# Autodesk Inventor assembly: Estante
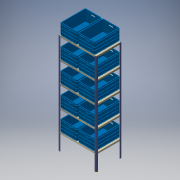
[picture p0: Inventor's stored thumbnail of the model, 180x180]
Saved by Autodesk Inventor 2016 (Build 200138000, 138)
## iProperties
Created: 2015-11-12
Part Number: Estante
Material: Genérico
Document SubType Name: Assembly
Designer: David
_SolveAssemblyDoc: Frame Generator Solve Assembly
_Version: 15.0.0
Author: David
## Documents named in this file (6)
- D:\Programas\xampp\htdocs\localUnal\storage\macros\cuarto\Modelado\estantería\Estantes Grandes\Estante.iam
- D:\Programas\xampp\htdocs\localUnal\storage\macros\cuarto\Modelado\estantería\estantería\Esqueleto.ipt
- D:\Programas\xampp\htdocs\localUnal\storage\macros\cuarto\Modelado\estantería\Estantes Grandes\Estante1\Frame\Frame0001.iam
- D:\Programas\xampp\htdocs\localUnal\storage\macros\cuarto\Modelado\estantería\estantería\lámina.ipt
- D:\Programas\xampp\htdocs\localUnal\storage\macros\cuarto\Modelado\estantería\estantería\HBOLT 0.2500-20x1x0.75-S.ipt
- D:\Programas\xampp\htdocs\localUnal\storage\macros\cuarto\Modelado\estantería\Storage Bin 50L.ipt
## Components (37 placed, 5 different names)
1. Esqueleto:1
2. Frame0001:1 [sub-assembly] — Nivelación:1, Coincidencia:1, Insertar:1, Coincidencia:2, Coincidencia:3, Coincidencia:4, Coincidencia:5, Coincidencia:6, Coincidencia:7, Coincidencia:8, Coincidencia:9, Coincidencia:10, Coincidencia:11, Coincidencia:12, Coincidencia:13, Coincidencia:14, Coincidencia:15, Coincidencia:16, Coincidencia:17, Coincidencia:18, Coincidencia:19, Coincidencia:20, Coincidencia:21, Coincidencia:22, Coincidencia:23, Coincidencia:24, Coincidencia:25, Coincidencia:26, Coincidencia:27, Coincidencia:28, Coincidencia:29, Coincidencia:30, Coincidencia:31, Coincidencia:32, Coincidencia:33, Coincidencia:34, Coincidencia:35, Coincidencia:36, Coincidencia:37, Coincidencia:38, Coincidencia:39, Coincidencia:41, Nivelación:14, Coincidencia:43
3. lámina:1 — Nivelación:1, Nivelación:2, Nivelación:3, Nivelación:4, Coincidencia:40, Coincidencia:42
4. lámina:2 — Nivelación:11, Nivelación:12, Nivelación:13
5. lámina:3 — Nivelación:5, Nivelación:6, Nivelación:7, Nivelación:8, Nivelación:9, Nivelación:10
6. lámina:4 — Nivelación:8, Nivelación:9, Nivelación:10, Nivelación:12, Nivelación:13
7. lámina:5 — Nivelación:2, Nivelación:3, Nivelación:4, Nivelación:5, Nivelación:6, Nivelación:7, Nivelación:11
8. HBOLT 0.2500-20x1x0.75-S:1 — Coincidencia:1, Insertar:1
9. HBOLT 0.2500-20x1x0.75-S:2 — Coincidencia:10, Coincidencia:16
10. HBOLT 0.2500-20x1x0.75-S:3 — Coincidencia:2, Coincidencia:6
11. HBOLT 0.2500-20x1x0.75-S:4 — Coincidencia:11, Coincidencia:19
12. HBOLT 0.2500-20x1x0.75-S:5 — Coincidencia:3, Coincidencia:9
13. HBOLT 0.2500-20x1x0.75-S:6 — Coincidencia:12, Coincidencia:17
14. HBOLT 0.2500-20x1x0.75-S:7 — Coincidencia:4, Coincidencia:7
15. HBOLT 0.2500-20x1x0.75-S:8 — Coincidencia:13, Coincidencia:18
16. HBOLT 0.2500-20x1x0.75-S:9 — Coincidencia:5, Coincidencia:8
17. HBOLT 0.2500-20x1x0.75-S:10 — Coincidencia:14, Coincidencia:15
18. HBOLT 0.2500-20x1x0.75-S:11 — Coincidencia:20, Coincidencia:26
19. HBOLT 0.2500-20x1x0.75-S:12 — Coincidencia:22, Coincidencia:27
20. HBOLT 0.2500-20x1x0.75-S:13 — Coincidencia:32, Coincidencia:35
21. HBOLT 0.2500-20x1x0.75-S:14 — Coincidencia:21, Coincidencia:28
22. HBOLT 0.2500-20x1x0.75-S:15 — Coincidencia:34, Coincidencia:38
23. HBOLT 0.2500-20x1x0.75-S:16 — Coincidencia:24, Coincidencia:29
24. HBOLT 0.2500-20x1x0.75-S:17 — Coincidencia:30, Coincidencia:37
25. HBOLT 0.2500-20x1x0.75-S:18 — Coincidencia:31, Coincidencia:39
26. HBOLT 0.2500-20x1x0.75-S:19 — Coincidencia:33, Coincidencia:36
27. HBOLT 0.2500-20x1x0.75-S:20 — Coincidencia:23, Coincidencia:25
28. Storage Bin 50L:2 — Nivelación:15, Coincidencia:42, Coincidencia:43
29. Storage Bin 50L:1 — Coincidencia:40, Coincidencia:41, Nivelación:14, Nivelación:15
30. Storage Bin 50L:3
31. Storage Bin 50L:4
32. Storage Bin 50L:5
33. Storage Bin 50L:6
34. Storage Bin 50L:7
35. Storage Bin 50L:8
36. Storage Bin 50L:9
37. Storage Bin 50L:10
## Component patterns: (5 elements, first: Storage Bin 50L:2 + Storage Bin 50L:1)
## Relationships (59: Mate 43, Flush 15, Insert 1)
- Nivelación:1 [Flush]: Frame0001:1 ↔ lámina:1
- Nivelación:2 [Flush] (500 mm): lámina:1 ↔ lámina:5
- Nivelación:3 [Flush]: lámina:1 ↔ lámina:5
- Nivelación:4 [Flush]: lámina:1 ↔ lámina:5
- Nivelación:5 [Flush]: lámina:3 ↔ lámina:5
- Nivelación:6 [Flush] (500 mm): lámina:3 ↔ lámina:5
- Nivelación:7 [Flush]: lámina:3 ↔ lámina:5
- Nivelación:8 [Flush] (500 mm): lámina:3 ↔ lámina:4
- Nivelación:9 [Flush]: lámina:3 ↔ lámina:4
- Nivelación:10 [Flush]: lámina:3 ↔ lámina:4
- Nivelación:11 [Flush]: lámina:2 ↔ lámina:5
- Nivelación:12 [Flush] (500 mm): lámina:2 ↔ lámina:4
- Nivelación:13 [Flush]: lámina:2 ↔ lámina:4
- Coincidencia:1 [Mate]: Frame0001:1 ↔ HBOLT 0.2500-20x1x0.75-S:1
- Insertar:1: Frame0001:1 ↔ HBOLT 0.2500-20x1x0.75-S:1
- Coincidencia:2 [Mate]: Frame0001:1 ↔ HBOLT 0.2500-20x1x0.75-S:3
- Coincidencia:3 [Mate]: Frame0001:1 ↔ HBOLT 0.2500-20x1x0.75-S:5
- Coincidencia:4 [Mate]: Frame0001:1 ↔ HBOLT 0.2500-20x1x0.75-S:7
- Coincidencia:5 [Mate]: Frame0001:1 ↔ HBOLT 0.2500-20x1x0.75-S:9
- Coincidencia:6 [Mate]: Frame0001:1 ↔ HBOLT 0.2500-20x1x0.75-S:3
- Coincidencia:7 [Mate]: Frame0001:1 ↔ HBOLT 0.2500-20x1x0.75-S:7
- Coincidencia:8 [Mate]: Frame0001:1 ↔ HBOLT 0.2500-20x1x0.75-S:9
- Coincidencia:9 [Mate]: Frame0001:1 ↔ HBOLT 0.2500-20x1x0.75-S:5
- Coincidencia:10 [Mate]: Frame0001:1 ↔ HBOLT 0.2500-20x1x0.75-S:2
- Coincidencia:11 [Mate]: Frame0001:1 ↔ HBOLT 0.2500-20x1x0.75-S:4
- Coincidencia:12 [Mate]: Frame0001:1 ↔ HBOLT 0.2500-20x1x0.75-S:6
- Coincidencia:13 [Mate]: Frame0001:1 ↔ HBOLT 0.2500-20x1x0.75-S:8
- Coincidencia:14 [Mate]: Frame0001:1 ↔ HBOLT 0.2500-20x1x0.75-S:10
- Coincidencia:15 [Mate]: Frame0001:1 ↔ HBOLT 0.2500-20x1x0.75-S:10
- Coincidencia:16 [Mate]: Frame0001:1 ↔ HBOLT 0.2500-20x1x0.75-S:2
- Coincidencia:17 [Mate]: Frame0001:1 ↔ HBOLT 0.2500-20x1x0.75-S:6
- Coincidencia:18 [Mate]: Frame0001:1 ↔ HBOLT 0.2500-20x1x0.75-S:8
- Coincidencia:19 [Mate]: Frame0001:1 ↔ HBOLT 0.2500-20x1x0.75-S:4
- Coincidencia:20 [Mate]: Frame0001:1 ↔ HBOLT 0.2500-20x1x0.75-S:11
- Coincidencia:21 [Mate]: Frame0001:1 ↔ HBOLT 0.2500-20x1x0.75-S:14
- Coincidencia:22 [Mate]: Frame0001:1 ↔ HBOLT 0.2500-20x1x0.75-S:12
- Coincidencia:23 [Mate]: Frame0001:1 ↔ HBOLT 0.2500-20x1x0.75-S:20
- Coincidencia:24 [Mate]: Frame0001:1 ↔ HBOLT 0.2500-20x1x0.75-S:16
- Coincidencia:25 [Mate]: Frame0001:1 ↔ HBOLT 0.2500-20x1x0.75-S:20
- Coincidencia:26 [Mate]: Frame0001:1 ↔ HBOLT 0.2500-20x1x0.75-S:11
- Coincidencia:27 [Mate]: Frame0001:1 ↔ HBOLT 0.2500-20x1x0.75-S:12
- Coincidencia:28 [Mate]: Frame0001:1 ↔ HBOLT 0.2500-20x1x0.75-S:14
- Coincidencia:29 [Mate]: Frame0001:1 ↔ HBOLT 0.2500-20x1x0.75-S:16
- Coincidencia:30 [Mate]: Frame0001:1 ↔ HBOLT 0.2500-20x1x0.75-S:17
- Coincidencia:31 [Mate]: Frame0001:1 ↔ HBOLT 0.2500-20x1x0.75-S:18
- Coincidencia:32 [Mate]: Frame0001:1 ↔ HBOLT 0.2500-20x1x0.75-S:13
- Coincidencia:33 [Mate]: Frame0001:1 ↔ HBOLT 0.2500-20x1x0.75-S:19
- Coincidencia:34 [Mate]: Frame0001:1 ↔ HBOLT 0.2500-20x1x0.75-S:15
- Coincidencia:35 [Mate]: Frame0001:1 ↔ HBOLT 0.2500-20x1x0.75-S:13
- Coincidencia:36 [Mate]: Frame0001:1 ↔ HBOLT 0.2500-20x1x0.75-S:19
- Coincidencia:37 [Mate]: Frame0001:1 ↔ HBOLT 0.2500-20x1x0.75-S:17
- Coincidencia:38 [Mate]: Frame0001:1 ↔ HBOLT 0.2500-20x1x0.75-S:15
- Coincidencia:39 [Mate]: Frame0001:1 ↔ HBOLT 0.2500-20x1x0.75-S:18
- Coincidencia:40 [Mate]: lámina:1 ↔ Storage Bin 50L:1
- Coincidencia:41 [Mate]: Frame0001:1 ↔ Storage Bin 50L:1
- Nivelación:14 [Flush]: Frame0001:1 ↔ Storage Bin 50L:1
- Nivelación:15 [Flush]: Storage Bin 50L:2 ↔ Storage Bin 50L:1
- Coincidencia:42 [Mate]: lámina:1 ↔ Storage Bin 50L:2
- Coincidencia:43 [Mate]: Frame0001:1 ↔ Storage Bin 50L:2
